# Autodesk Inventor assembly: Funnel
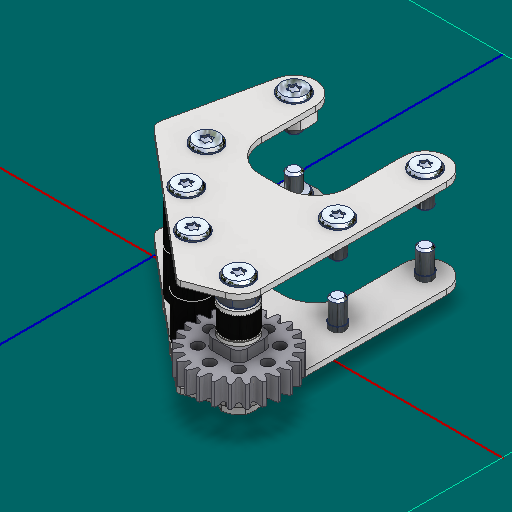
[picture p0: Inventor's stored thumbnail of the model, 512x512]
Saved by Autodesk Inventor 2025 (Build 290162000, 162)
## iProperties
Created: 2024-10-18
Part Number: Funnel
Document SubType Name: Assembly
Designer: averey
Author: averey
## Documents named in this file (18)
- C:\Users\avere\VEX\High Stakes\CAD\V2\Chassis\Drivebay Left\Funnel.iam
- C:\Users\avere\VEX\High Stakes\CAD\V2\Chassis\Drivebay Left\Custom Parts\Funnel Gusset.ipt
- C:\Users\avere\VEX\High Stakes\CAD\ROBOPROS-CAD-Inventor\Motion\Spacers\Spacer Nylon .375 OD\NSpacer .375 OD x .500.ipt
- C:\Users\avere\VEX\High Stakes\CAD\ROBOPROS-CAD-Inventor\Motion\Spacers\Spacer Nylon .375 OD.ipt
- C:\Users\avere\VEX\High Stakes\CAD\ROBOPROS-CAD-Inventor\Structure\Hardware\Screw Steel - Star\SScrew Star Smooth 1.250.ipt
- C:\Users\avere\VEX\High Stakes\CAD\ROBOPROS-CAD-Inventor\Structure\Hardware\Screw Steel - Star.ipt
- C:\Users\avere\VEX\High Stakes\CAD\ROBOPROS-CAD-Inventor\Structure\Hardware\Nut Nylon\Nut Nylon - White.ipt
- C:\Users\avere\VEX\High Stakes\CAD\ROBOPROS-CAD-Inventor\Structure\Hardware\Nut Nylon.ipt
- C:\Users\avere\VEX\High Stakes\CAD\ROBOPROS-CAD-Inventor\Structure\Hardware\Screw Shoulder Robosource\SScrew Shoulder Smooth .375 x .12.ipt
- C:\Users\avere\VEX\High Stakes\CAD\ROBOPROS-CAD-Inventor\Structure\Hardware\Screw Shoulder Robosource.ipt
- C:\Users\avere\VEX\High Stakes\CAD\ROBOPROS-CAD-Inventor\Modified Parts\Half Cut HS 24T Gear, No Insert.ipt
- C:\Users\avere\VEX\High Stakes\CAD\ROBOPROS-CAD-Inventor\Structure\Hardware\Nut Keps.ipt
- C:\Users\avere\VEX\High Stakes\CAD\ROBOPROS-CAD-Inventor\Motion\Spacers\Spacer Nylon .375 OD\NSpacer .375 OD x .250.ipt
- C:\Users\avere\VEX\High Stakes\CAD\ROBOPROS-CAD-Inventor\Motion\Spacers\Washer Teflon\TWasher .375 OD x .04000.ipt
- C:\Users\avere\VEX\High Stakes\CAD\ROBOPROS-CAD-Inventor\Motion\Spacers\Washer Steel\SWasher .375 OD x .015625.ipt
- C:\Users\avere\VEX\High Stakes\CAD\ROBOPROS-CAD-Inventor\Structure\Hardware\Screw Shoulder Robosource\SScrew Shoulder Smooth .290 x .09.ipt
- C:\Users\avere\VEX\High Stakes\CAD\ROBOPROS-CAD-Inventor\Motion\Spacers\Washer Teflon.ipt
- C:\Users\avere\VEX\High Stakes\CAD\ROBOPROS-CAD-Inventor\Motion\Spacers\Washer Steel.ipt
## Components (30 placed, 11 different names)
1. Funnel Gusset:1 — Insert:4, Insert:5, Insert:6, Insert:9, Insert:14, Insert:20, Insert:22, Insert:23
2. Funnel Gusset:2 — Insert:2, Insert:7, Insert:8, Insert:10, Insert:12, Insert:13, Insert:19, Insert:21
3. NSpacer .375 OD x .500:1 — Insert:1
4. NSpacer .375 OD x .500:2 — Insert:1, Insert:2
5. NSpacer .375 OD x .500:3 — Insert:4
6. NSpacer .375 OD x .500:4
7. SScrew Star Smooth 1.250:1 — Insert:5
8. SScrew Star Smooth 1.250:2 — Insert:6
9. Nut Nylon - White:1 — Insert:8
10. Nut Nylon - White:2 — Insert:7
11. Nut Nylon - White:3 — Insert:12
12. Half Cut HS 24T Gear, No Insert:1 — Insert:13, Insert:18
13. Nut Keps:1 — Insert:14
14. NSpacer .375 OD x .250:5 — Insert:15, Insert:16
15. TWasher .375 OD x .04000:1 — Insert:17, Insert:18
16. TWasher .375 OD x .04000:2 — Insert:15
17. SWasher .375 OD x .015625:1 — Insert:16, Insert:17
18. SScrew Star Smooth 1.250:3 — Insert:20
19. Nut Nylon - White:4 — Insert:19
20. SScrew Shoulder Smooth .290 x .09:9 — Insert:21
21. Nut Nylon - White:5 — Insert:22
22. SScrew Shoulder Smooth .290 x .09:10 — Insert:23
23. SScrew Shoulder Smooth .375 x .12:1 — Insert:9
24. SScrew Shoulder Smooth .375 x .12:2
25. SScrew Shoulder Smooth .375 x .12:3
26. SScrew Shoulder Smooth .375 x .12:4
27. SScrew Shoulder Smooth .375 x .12:5 — Insert:10
28. SScrew Shoulder Smooth .375 x .12:6
29. SScrew Shoulder Smooth .375 x .12:7
30. SScrew Shoulder Smooth .375 x .12:8
## Component patterns: Top Mounting Screws (4 elements), Bottom Mounting Screw Pattern (4 elements)
## Relationships (23: Insert 22, Mate 1)
- [Mate]: Funnel Gusset:1 ↔ Funnel Gusset:2
- Insert:1: NSpacer .375 OD x .500:1 ↔ NSpacer .375 OD x .500:2
- Insert:2: Funnel Gusset:2 ↔ NSpacer .375 OD x .500:2
- [Insert]: NSpacer .375 OD x .500:3 ↔ NSpacer .375 OD x .500:4
- Insert:4: Funnel Gusset:1 ↔ NSpacer .375 OD x .500:3
- Insert:5: Funnel Gusset:1 ↔ SScrew Star Smooth 1.250:1
- Insert:6: Funnel Gusset:1 ↔ SScrew Star Smooth 1.250:2
- Insert:7: Funnel Gusset:2 ↔ Nut Nylon - White:2
- Insert:8: Funnel Gusset:2 ↔ Nut Nylon - White:1
- Insert:9: Funnel Gusset:1 ↔ SScrew Shoulder Smooth .375 x .12:1
- Insert:10: Funnel Gusset:2 ↔ SScrew Shoulder Smooth .375 x .12:5
- Insert:12: Funnel Gusset:2 ↔ Nut Nylon - White:3
- Insert:13: Funnel Gusset:2 ↔ Half Cut HS 24T Gear, No Insert:1
- Insert:14: Funnel Gusset:1 ↔ Nut Keps:1
- Insert:15: NSpacer .375 OD x .250:5 ↔ TWasher .375 OD x .04000:2
- Insert:16: NSpacer .375 OD x .250:5 ↔ SWasher .375 OD x .015625:1
- Insert:17: TWasher .375 OD x .04000:1 ↔ SWasher .375 OD x .015625:1
- Insert:18: Half Cut HS 24T Gear, No Insert:1 ↔ TWasher .375 OD x .04000:1
- Insert:19: Funnel Gusset:2 ↔ Nut Nylon - White:4
- Insert:20: Funnel Gusset:1 ↔ SScrew Star Smooth 1.250:3
- Insert:21 (1.5875 mm): Funnel Gusset:2 ↔ SScrew Shoulder Smooth .290 x .09:9
- Insert:22 (1.5875 mm): Funnel Gusset:1 ↔ Nut Nylon - White:5
- Insert:23: Funnel Gusset:1 ↔ SScrew Shoulder Smooth .290 x .09:10
## Named parameters: d3_d1 = 0 mm
